# Autodesk Inventor assembly: Assemblybridge
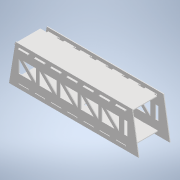
[picture p0: Inventor's stored thumbnail of the model, 180x180]
Saved by Autodesk Inventor 2022 (Build 260153000, 153)
## iProperties
Created: 2022-03-08
Part Number: Assemblybridge
Document SubType Name: Assembly
Designer: anjarwala7025
Author: anjarwala7025
## Documents named in this file (4)
- H:\Assemblybridge.iam
- H:\Bridge.ipt
- H:\BridgeBottom.ipt
- H:\BridgeRoof.ipt
## Components (4 placed, 3 different names)
1. Bridge:1 — Mate:3
2. Bridge:2 — Mate:1, Mate:2
3. BridgeBottom:1 — Mate:2
4. BridgeRoof:1 — Mate:1, Mate:3
## Relationships (3: Mate 3)
- Mate:1: Bridge:2 ↔ BridgeRoof:1
- Mate:2: Bridge:2 ↔ BridgeBottom:1
- Mate:3: Bridge:1 ↔ BridgeRoof:1
